# Autodesk Inventor assembly: Estructura
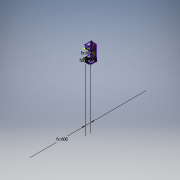
[picture p0: Inventor's stored thumbnail of the model, 180x180]
Saved by Autodesk Inventor 2018 (Build 220112000, 112)
## iProperties
Created: 2018-06-23
Part Number: Estructura
Document SubType Name: Assembly
Designer: sebas
_SolveAssemblyDoc: Frame Generator Solve Assembly
_Version: 15.0.0
Author: sebas
## Documents named in this file (4)
- C:\Users\sebas\OneDrive\Documents\Inventor\Escritorio\Estructura.iam
- C:\Users\sebas\OneDrive\Documents\Inventor\Escritorio\Esqueleto.ipt
- C:\Users\sebas\OneDrive\Documents\Inventor\Escritorio\Estructura\Frame\Frame0001.iam
- C:\Users\sebas\OneDrive\Documents\Inventor\Escritorio\Tabla.ipt
## Components (3 placed, 3 different names)
1. Esqueleto:1 — Mate:1, Mate:2
2. Frame0001:1 [sub-assembly]
3. Tabla:1 — Mate:1, Mate:2
## Relationships (2: Mate 2)
- Mate:1: Esqueleto:1 ↔ Tabla:1
- Mate:2: Esqueleto:1 ↔ Tabla:1
